# Autodesk Inventor assembly: HexTrayRed
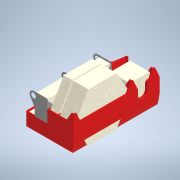
[picture p0: Inventor's stored thumbnail of the model, 180x180]
Saved by Autodesk Inventor 2021 (Build 250183000, 183)
## iProperties
Created: 2023-03-18
Part Number: HexTrayRed
Document SubType Name: Assembly
Designer: Bradley
Author: Bradley
## Documents named in this file (13)
- C:\Users\Bradley\Git\TI4\Hexes\HexTrayRed.iam
- C:\Users\Bradley\Git\TI4\Components\Hex_Hyperlanes_All.ipt
- C:\Users\Bradley\Git\TI4\Components\Hex_Mecatol.ipt
- C:\Users\Bradley\Git\TI4\Components\Hex_Reds_All.ipt
- C:\Users\Bradley\Git\TI4\Hexes\HexTrayRed.ipt
- C:\Users\Bradley\Git\TI4\Components\ActionCards_All.ipt
- C:\Users\Bradley\Git\TI4\Components\Exploration_SingleType.ipt
- C:\Users\Bradley\Git\TI4\Components\Objects_Public_SingleType.ipt
- C:\Users\Bradley\Git\TI4\Components\Objects_Secret_All.ipt
- C:\Users\Bradley\Git\TI4\Components\Relics_All.ipt
- C:\Users\Bradley\Git\TI4\Components\Planets_All.ipt
- C:\Users\Bradley\Git\TI4\Components\Agendas_All.ipt
- C:\Users\Bradley\Git\TI4\Hexes\HexTrayRed_Insert.ipt
## Components (20 placed, 12 different names)
1. Hex_Hyperlanes_All:1 — Mate:1, Flush:1, Flush:2, Flush:4, Flush:5, Mate:4
2. Hex_Mecatol:1 — Mate:1, Flush:1, Flush:2
3. Hex_Reds_All:1 — Mate:2, Mate:3, Flush:3, Flush:4, Flush:5
4. HexTrayRed:1 — Mate:2, Mate:3, Flush:3, Mate:4, Mate:11, Mate:12, Mate:13, Mate:16, Mate:17, Mate:18, Mate:19, Mate:20, Mate:21, Mate:22, Mate:23, Mate:24, Mate:25, Mate:26, Mate:27, Mate:28, Mate:29, Mate:30, Mate:31, Mate:32, Mate:33, Flush:20, Mate:34
5. ActionCards_All:1 — Mate:19, Mate:20, Mate:21
6. Exploration_SingleType:1 — Mate:11, Mate:12, Mate:13
7. Exploration_SingleType:2
8. Exploration_SingleType:3
9. Exploration_SingleType:4
10. Objects_Public_SingleType:1 — Mate:16, Mate:17, Mate:18
11. Objects_Public_SingleType:2
12. Objects_Secret_All:1
13. Exploration_SingleType:5 — Mate:22, Mate:23, Mate:24, Flush:16
14. Exploration_SingleType:6 — Mate:25, Mate:26, Flush:16, Flush:17
15. Exploration_SingleType:7 — Mate:27, Mate:28, Flush:17, Flush:18
16. Exploration_SingleType:8 — Mate:29, Mate:30, Flush:18, Flush:19
17. Relics_All:1 — Mate:31, Mate:32, Flush:19
18. Planets_All:1 — Mate:35, Mate:38, Mate:40
19. Agendas_All:1 — Mate:36, Mate:37, Mate:39
20. HexTrayRed_Insert:1 — Mate:33, Flush:20, Mate:34, Mate:35, Mate:36, Mate:37, Mate:38, Mate:39, Mate:40
## Relationships (57: Mate 37, Flush 20)
- Mate:1: Hex_Hyperlanes_All:1 ↔ Hex_Mecatol:1
- Flush:1: Hex_Hyperlanes_All:1 ↔ Hex_Mecatol:1
- Flush:2: Hex_Hyperlanes_All:1 ↔ Hex_Mecatol:1
- Mate:2 (0.3 mm): Hex_Reds_All:1 ↔ HexTrayRed:1
- Mate:3: Hex_Reds_All:1 ↔ HexTrayRed:1
- Flush:3: Hex_Reds_All:1 ↔ HexTrayRed:1
- Flush:4: Hex_Hyperlanes_All:1 ↔ Hex_Reds_All:1
- Flush:5: Hex_Hyperlanes_All:1 ↔ Hex_Reds_All:1
- Mate:4 (0.4 mm): Hex_Hyperlanes_All:1 ↔ HexTrayRed:1
- [Mate]: Exploration_SingleType:1 ↔ Exploration_SingleType:2
- [Mate]: Exploration_SingleType:2 ↔ Exploration_SingleType:3
- [Mate]: Exploration_SingleType:3 ↔ Exploration_SingleType:4
- [Flush]: Exploration_SingleType:3 ↔ Exploration_SingleType:4
- [Flush]: Exploration_SingleType:2 ↔ Exploration_SingleType:3
- [Flush]: Exploration_SingleType:1 ↔ Exploration_SingleType:2
- [Flush]: Exploration_SingleType:3 ↔ Exploration_SingleType:4
- [Flush]: Exploration_SingleType:2 ↔ Exploration_SingleType:3
- [Flush]: Exploration_SingleType:1 ↔ Exploration_SingleType:2
- Mate:11: HexTrayRed:1 ↔ Exploration_SingleType:1
- Mate:12 (0.5 mm): HexTrayRed:1 ↔ Exploration_SingleType:1
- Mate:13 (0.5 mm): HexTrayRed:1 ↔ Exploration_SingleType:1
- [Mate]: Objects_Public_SingleType:1 ↔ Objects_Public_SingleType:2
- [Mate]: Objects_Public_SingleType:2 ↔ Objects_Secret_All:1
- [Flush]: Objects_Public_SingleType:2 ↔ Objects_Secret_All:1
- [Flush]: Objects_Public_SingleType:1 ↔ Objects_Public_SingleType:2
- [Flush]: Objects_Public_SingleType:1 ↔ Objects_Public_SingleType:2
- [Flush]: Objects_Public_SingleType:2 ↔ Objects_Secret_All:1
- Mate:16: HexTrayRed:1 ↔ Objects_Public_SingleType:1
- Mate:17 (0.5 mm): HexTrayRed:1 ↔ Objects_Public_SingleType:1
- Mate:18 (0.5 mm): HexTrayRed:1 ↔ Objects_Public_SingleType:1
- Mate:19: HexTrayRed:1 ↔ ActionCards_All:1
- Mate:20 (0.5 mm): HexTrayRed:1 ↔ ActionCards_All:1
- Mate:21 (0.5 mm): HexTrayRed:1 ↔ ActionCards_All:1
- Mate:22: HexTrayRed:1 ↔ Exploration_SingleType:5
- Mate:23: HexTrayRed:1 ↔ Exploration_SingleType:5
- Mate:24 (0.5 mm): HexTrayRed:1 ↔ Exploration_SingleType:5
- Mate:25: HexTrayRed:1 ↔ Exploration_SingleType:6
- Mate:26: HexTrayRed:1 ↔ Exploration_SingleType:6
- Mate:27: HexTrayRed:1 ↔ Exploration_SingleType:7
- Mate:28: HexTrayRed:1 ↔ Exploration_SingleType:7
- Mate:29: HexTrayRed:1 ↔ Exploration_SingleType:8
- Mate:30: HexTrayRed:1 ↔ Exploration_SingleType:8
- Flush:16: Exploration_SingleType:5 ↔ Exploration_SingleType:6
- Flush:17: Exploration_SingleType:6 ↔ Exploration_SingleType:7
- Flush:18: Exploration_SingleType:7 ↔ Exploration_SingleType:8
- Mate:31: HexTrayRed:1 ↔ Relics_All:1
- Mate:32: HexTrayRed:1 ↔ Relics_All:1
- Flush:19: Exploration_SingleType:8 ↔ Relics_All:1
- Mate:33: HexTrayRed:1 ↔ HexTrayRed_Insert:1
- Flush:20: HexTrayRed:1 ↔ HexTrayRed_Insert:1
- Mate:34: HexTrayRed:1 ↔ HexTrayRed_Insert:1
- Mate:35: Planets_All:1 ↔ HexTrayRed_Insert:1
- Mate:36: Agendas_All:1 ↔ HexTrayRed_Insert:1
- Mate:37: Agendas_All:1 ↔ HexTrayRed_Insert:1
- Mate:38: Planets_All:1 ↔ HexTrayRed_Insert:1
- Mate:39 (0.5 mm): Agendas_All:1 ↔ HexTrayRed_Insert:1
- Mate:40 (0.5 mm): Planets_All:1 ↔ HexTrayRed_Insert:1
